# Autodesk Inventor assembly: Xaxis_VarB
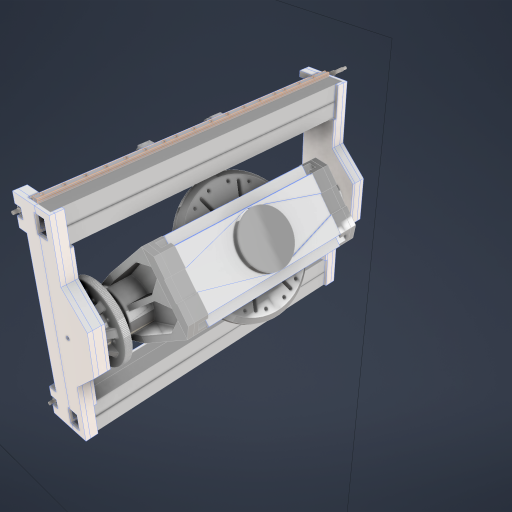
[picture p0: Inventor's stored thumbnail of the model, 512x512]
Saved by Autodesk Inventor 2024 (Build 280153000, 153)
## iProperties
Created: 2023-03-08
Part Number: Xaxis_VarB
Document SubType Name: Assembly
Designer: KirikDK
Mass: 76931.8 g
Surface Area: 63062.9 cm^2
Volume: 32523.9 cm^3
Density: 2.36539 g/cm^3
Author: KirikDK
## Documents named in this file (12)
- C:\Users\KirikDK\Documents\Stanok2023\Xaxis_VarB.iam
- C:\Users\KirikDK\Documents\Stanok2023\RailBlock.iam
- C:\Users\KirikDK\Documents\Stanok2023\TopZakrivka.ipt
- C:\Users\KirikDK\Documents\Stanok2023\SfuObrezki\SFU1605-600start.ipt
- C:\Users\KirikDK\Documents\Stanok2023\BF12 v1.ipt
- C:\Users\KirikDK\Documents\Stanok2023\BK12 v1.ipt
- C:\Users\KirikDK\Documents\Stanok2023\FlanecX_Aax_VarB.ipt
- C:\Users\KirikDK\Documents\Stanok2023\XAxisCreplCaretki.ipt
- C:\Users\KirikDK\Documents\Stanok2023\Aaxis_Ass.iam
- C:\Users\KirikDK\Documents\Stanok2023\nut housing v2.ipt
- C:\Users\KirikDK\Documents\Stanok2023\nut v3.ipt
- C:\Users\KirikDK\Documents\Stanok2023\A_axisShesterna.ipt
## Components (27 placed, 11 different names)
1. RailBlock:2 [sub-assembly] — Mate:13, Mate:14, Mate:15, Mate:20, Mate:21, Mate:36, Flush:2
2. RailBlock:3 [sub-assembly] — Mate:16, Mate:17, Mate:18, Mate:19, Mate:34, Flush:1
3. SFU1605-600start:1 — Mate:11, Mate:12, Mate:41, Mate:56, Mate:68
4. SFU1605-600start:2 — Mate:11, Mate:12, Mate:42, Mate:43
5. BF12 v1:1 — Mate:31, Mate:32
6. BK12 v1:1 — Mate:25, Mate:27, Mate:44, Mate:45, Mate:50
7. BF12 v1:2 — Mate:28, Mate:29, Mate:41
8. BK12 v1:2 — Mate:22, Mate:24, Mate:42, Mate:43, Mate:51
9. TopZakrivka:3 — Mate:34, Flush:1, Mate:38
10. TopZakrivka:4 — Mate:36, Flush:2, Mate:37
11. FlanecX_Aax_VarB:4 — Mate:19, Mate:20, Mate:21, Mate:22, Mate:24, Mate:25, Mate:27, Mate:46, Flush:3, Flush:4, Mate:50, Mate:51
12. FlanecX_Aax_VarB:5 — Mate:13, Mate:14, Mate:15, Mate:16, Mate:17, Mate:18, Mate:28, Mate:29, Mate:31, Mate:32, Mate:37, Mate:38, Mate:47, Flush:5, Flush:6
13. SFU1605-600start:3 — Mate:57, Mate:62
14. SFU1605-600start:4 — Mate:44, Mate:45
15. XAxisCreplCaretki:1 — Mate:46, Flush:3, Flush:4, Mate:48, Mate:49
16. XAxisCreplCaretki:2 — Mate:47, Flush:5, Flush:6
17. Aaxis_Ass:1 [sub-assembly] — Mate:48, Mate:49, Mate:71
18. nut housing v2:1 — Mate:52, Mate:55
19. nut housing v2:2 — Mate:53, Mate:54
20. nut v3:1 — Mate:53, Mate:54, Mate:56
21. nut v3:2 — Mate:52, Mate:55, Mate:57
22. nut housing v2:4
23. nut v3:4 — Mate:62
24. nut housing v2:6
25. nut v3:6 — Mate:68
26. A_axisShesterna:1 — Mate:69, Mate:70, Mate:71
27. A_axisShesterna:2 — Mate:69, Mate:70
## Relationships (57: Mate 51, Flush 6)
- Mate:11: SFU1605-600start:1 ↔ SFU1605-600start:2
- Mate:12: SFU1605-600start:1 ↔ SFU1605-600start:2
- Mate:13: RailBlock:2 ↔ FlanecX_Aax_VarB:5
- Mate:14: RailBlock:2 ↔ FlanecX_Aax_VarB:5
- Mate:15: RailBlock:2 ↔ FlanecX_Aax_VarB:5
- Mate:16: RailBlock:3 ↔ FlanecX_Aax_VarB:5
- Mate:17: RailBlock:3 ↔ FlanecX_Aax_VarB:5
- Mate:18: RailBlock:3 ↔ FlanecX_Aax_VarB:5
- Mate:19: RailBlock:3 ↔ FlanecX_Aax_VarB:4
- Mate:20: RailBlock:2 ↔ FlanecX_Aax_VarB:4
- Mate:21: RailBlock:2 ↔ FlanecX_Aax_VarB:4
- Mate:22: BK12 v1:2 ↔ FlanecX_Aax_VarB:4
- Mate:24: BK12 v1:2 ↔ FlanecX_Aax_VarB:4
- Mate:25: BK12 v1:1 ↔ FlanecX_Aax_VarB:4
- Mate:27: BK12 v1:1 ↔ FlanecX_Aax_VarB:4
- Mate:28: BF12 v1:2 ↔ FlanecX_Aax_VarB:5
- Mate:29: BF12 v1:2 ↔ FlanecX_Aax_VarB:5
- Mate:31: BF12 v1:1 ↔ FlanecX_Aax_VarB:5
- Mate:32: BF12 v1:1 ↔ FlanecX_Aax_VarB:5
- Mate:34: RailBlock:3 ↔ TopZakrivka:3
- Flush:1: RailBlock:3 ↔ TopZakrivka:3
- Mate:36: RailBlock:2 ↔ TopZakrivka:4
- Flush:2: RailBlock:2 ↔ TopZakrivka:4
- Mate:37: TopZakrivka:4 ↔ FlanecX_Aax_VarB:5
- Mate:38: TopZakrivka:3 ↔ FlanecX_Aax_VarB:5
- [Mate]: SFU1605-600start:3 ↔ SFU1605-600start:4
- [Mate]: SFU1605-600start:3 ↔ SFU1605-600start:4
- Mate:41: SFU1605-600start:1 ↔ BF12 v1:2
- Mate:42: SFU1605-600start:2 ↔ BK12 v1:2
- Mate:43: SFU1605-600start:2 ↔ BK12 v1:2
- Mate:44: BK12 v1:1 ↔ SFU1605-600start:4
- Mate:45: BK12 v1:1 ↔ SFU1605-600start:4
- Mate:46: FlanecX_Aax_VarB:4 ↔ XAxisCreplCaretki:1
- Flush:3: FlanecX_Aax_VarB:4 ↔ XAxisCreplCaretki:1
- Flush:4: FlanecX_Aax_VarB:4 ↔ XAxisCreplCaretki:1
- Mate:47: FlanecX_Aax_VarB:5 ↔ XAxisCreplCaretki:2
- Flush:5: FlanecX_Aax_VarB:5 ↔ XAxisCreplCaretki:2
- Flush:6: FlanecX_Aax_VarB:5 ↔ XAxisCreplCaretki:2
- Mate:48: XAxisCreplCaretki:1 ↔ Aaxis_Ass:1
- Mate:49: XAxisCreplCaretki:1 ↔ Aaxis_Ass:1
- Mate:50: BK12 v1:1 ↔ FlanecX_Aax_VarB:4
- Mate:51: BK12 v1:2 ↔ FlanecX_Aax_VarB:4
- Mate:52: nut housing v2:1 ↔ nut v3:2
- Mate:53: nut housing v2:2 ↔ nut v3:1
- Mate:54: nut housing v2:2 ↔ nut v3:1
- Mate:55: nut housing v2:1 ↔ nut v3:2
- Mate:56: SFU1605-600start:1 ↔ nut v3:1
- Mate:57: SFU1605-600start:3 ↔ nut v3:2
- [Mate]: nut housing v2:4 ↔ nut v3:4
- [Mate]: nut housing v2:4 ↔ nut v3:4
- Mate:62: SFU1605-600start:3 ↔ nut v3:4
- [Mate]: nut housing v2:6 ↔ nut v3:6
- [Mate]: nut housing v2:6 ↔ nut v3:6
- Mate:68: SFU1605-600start:1 ↔ nut v3:6
- Mate:69: A_axisShesterna:1 ↔ A_axisShesterna:2
- Mate:70: A_axisShesterna:1 ↔ A_axisShesterna:2
- Mate:71: Aaxis_Ass:1 ↔ A_axisShesterna:1
## Named parameters: d75_d25 = 0 mm, d76_d26 = 0 mm, d147_d144_d135 = 0 mm, d148_d145_d138 = 0 mm, d153_d150_d135 = 0 mm, d154_d151_d138 = 0 mm
